# Autodesk Inventor assembly: pen
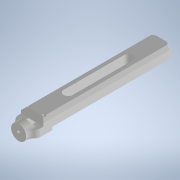
[picture p0: Inventor's stored thumbnail of the model, 180x180]
Saved by Autodesk Inventor 2020 (Build 240168000, 168)
## iProperties
Created: 2019-11-04
Part Number: pen
Document SubType Name: Assembly
Designer: psrob
Author: psrob
## Documents named in this file (3)
- E:\projects-2\haptic device gen3\hardware\pen.iam
- E:\projects-2\haptic device gen3\hardware\pen_1.ipt
- E:\projects-2\haptic device gen3\hardware\pen_2.ipt
## Components (2 placed, 2 different names)
1. pen_1:1 — Flush:1
2. pen_2:1 — Flush:1
## Relationships (1: Flush 1)
- Flush:1: pen_1:1 ↔ pen_2:1
